# Autodesk Inventor assembly: POM_T5_11
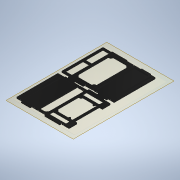
[picture p0: Inventor's stored thumbnail of the model, 180x180]
Saved by Autodesk Inventor 2020 (Build 240168000, 168)
## iProperties
Created: 2021-08-27
Part Number: POM_T5_11
Document SubType Name: Assembly
Designer: Masato
Author: Masato
## Documents named in this file (5)
- C:\Inventor\SUSTAINA-OP\Cam\POM_T5_11.iam
- C:\Inventor\SUSTAINA-OP\Cam\DisposableBoard.ipt
- C:\Inventor\SUSTAINA-OP\UpperBody\Cockpit\Cockpit_carrier_board_frame.ipt
- C:\Inventor\SUSTAINA-OP\UpperBody\Cockpit\Cockpit_circuit_board_frame.ipt
- C:\Inventor\SUSTAINA-OP\UpperBody\Cockpit\Cockpit_front_frame.ipt
## Components (5 placed, 4 different names)
1. DisposableBoard:1 — メイト:2, メイト:1, フラッシュ:1, フラッシュ:2, メイト:5, メイト:9, メイト:12, フラッシュ:3, フラッシュ:4, メイト:13
2. Cockpit_carrier_board_frame:1 — メイト:5, メイト:11, メイト:15, フラッシュ:6
3. Cockpit_circuit_board_frame:1 — メイト:10, フラッシュ:5, メイト:13, メイト:14
4. Cockpit_front_frame:1 — メイト:9, メイト:10, メイト:11
5. Cockpit_front_frame:2 — メイト:12, フラッシュ:3, フラッシュ:4, フラッシュ:5, メイト:14, メイト:15, フラッシュ:6
## Relationships (16: Mate 10, Flush 6)
- メイト:2 [Mate]: DisposableBoard:1
- メイト:1 [Mate]: DisposableBoard:1
- フラッシュ:1 [Flush]: DisposableBoard:1
- フラッシュ:2 [Flush]: DisposableBoard:1
- メイト:5 [Mate]: DisposableBoard:1 ↔ Cockpit_carrier_board_frame:1
- メイト:9 [Mate]: DisposableBoard:1 ↔ Cockpit_front_frame:1
- メイト:10 [Mate] (2.5 mm): Cockpit_circuit_board_frame:1 ↔ Cockpit_front_frame:1
- メイト:11 [Mate] (2.5 mm): Cockpit_carrier_board_frame:1 ↔ Cockpit_front_frame:1
- メイト:12 [Mate]: DisposableBoard:1 ↔ Cockpit_front_frame:2
- フラッシュ:3 [Flush] (2.5 mm): DisposableBoard:1 ↔ Cockpit_front_frame:2
- フラッシュ:4 [Flush] (2.5 mm): DisposableBoard:1 ↔ Cockpit_front_frame:2
- フラッシュ:5 [Flush]: Cockpit_circuit_board_frame:1 ↔ Cockpit_front_frame:2
- メイト:13 [Mate]: DisposableBoard:1 ↔ Cockpit_circuit_board_frame:1
- メイト:14 [Mate] (2.5 mm): Cockpit_circuit_board_frame:1 ↔ Cockpit_front_frame:2
- メイト:15 [Mate] (2.5 mm): Cockpit_carrier_board_frame:1 ↔ Cockpit_front_frame:2
- フラッシュ:6 [Flush]: Cockpit_carrier_board_frame:1 ↔ Cockpit_front_frame:2
